# Autodesk Inventor assembly: PortableVoltageStandard_Assembly
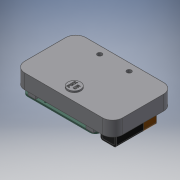
[picture p0: Inventor's stored thumbnail of the model, 180x180]
Saved by Autodesk Inventor 2019 (Build 230136000, 136)
## iProperties
Created: 2025-01-19
Part Number: PortableVoltageStandard_Assembly
Material: Générique
Document SubType Name: Assembly
Designer: Maxime
Author: Maxime
## iProperties of the stored document 9V-battery.ipt
Created: 2011-06-06
Part Number: 9V-battery
Material: Générique
Document SubType Name: Modeling
Designer: Maxime
Density: 1 g/cm^3
Appearance: Par défaut
Sending System: Kubotek KeyCreator 2011 V10.0.0 (21019)
Preprocessor: Spatial Interop R20 SP3
Title: icpv2
Author: keycreator
Revision Number: NONE
## Documents named in this file (7)
- **C:\Users\Maxime\Desktop\PROJETS\Portable-Voltage-Standard\mechanical\PortableVoltageStandard_Assembly.iam*LocalDocs*xMpgmies4P4ndeuk3V5evyuvlLh*9V-battery.ipt
- C:\Users\Maxime\Desktop\PROJETS\Portable-Voltage-Standard\mechanical\PortableVoltageStandard_Assembly.iam
- C:\Users\Maxime\Desktop\PROJETS\Portable-Voltage-Standard\mechanical\PCB.iam
- C:\Users\Maxime\Desktop\PROJETS\Portable-Voltage-Standard\mechanical\Case_Bottom.ipt
- C:\Users\Maxime\Desktop\PROJETS\Portable-Voltage-Standard\mechanical\Case_Top.ipt
- C:\Users\Maxime\Desktop\PROJETS\Portable-Voltage-Standard\mechanical\Power_Button.ipt
- C:\Users\Maxime\Desktop\PROJETS\Portable-Voltage-Standard\mechanical\9V-battery.stp
## Components (5 placed, 5 different names)
1. PCB:1 [sub-assembly] — Placage:1, Placage:2, Placage:3, Placage:10, Placage:11, Placage:12, Placage:13, Placage:14
2. 9V-battery:1 — Placage:6, Placage:7, Placage:8
3. Case_Bottom:1 — Placage:1, Placage:2, Placage:3, Placage:6, Placage:7, Placage:8, Placage:9
4. Case_Top:1 — Placage:9, Placage:10, Placage:11
5. Power_Button:1 — Placage:12, Placage:13, Placage:14
## Relationships (12: Mate 12)
- Placage:1 [Mate]: PCB:1 ↔ Case_Bottom:1
- Placage:2 [Mate]: PCB:1 ↔ Case_Bottom:1
- Placage:3 [Mate]: PCB:1 ↔ Case_Bottom:1
- Placage:6 [Mate] (0.15 mm): 9V-battery:1 ↔ Case_Bottom:1
- Placage:7 [Mate] (0.6 mm): 9V-battery:1 ↔ Case_Bottom:1
- Placage:8 [Mate] (0.15 mm): 9V-battery:1 ↔ Case_Bottom:1
- Placage:9 [Mate]: Case_Bottom:1 ↔ Case_Top:1
- Placage:10 [Mate]: PCB:1 ↔ Case_Top:1
- Placage:11 [Mate]: PCB:1 ↔ Case_Top:1
- Placage:12 [Mate]: PCB:1 ↔ Power_Button:1
- Placage:13 [Mate]: PCB:1 ↔ Power_Button:1
- Placage:14 [Mate]: PCB:1 ↔ Power_Button:1
